# Autodesk Inventor assembly: Lick
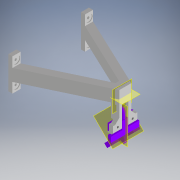
[picture p0: Inventor's stored thumbnail of the model, 180x180]
Saved by Autodesk Inventor 2020 (Build 240168000, 168)
## iProperties
Created: 2020-01-13
Part Number: Lick
Document SubType Name: Assembly
Designer: Knowblesse
Author: Knowblesse
## Documents named in this file (3)
- C:\VCF\Lobster\Apparatus\Lick\Lick.iam
- C:\VCF\Lobster\Apparatus\Lick\LickSensorMount_H.ipt
- C:\VCF\Lobster\Apparatus\Lick\LickModuleMount.ipt
## Components (2 placed, 2 different names)
1. LickSensorMount_H:1 — 강체:1
2. LickModuleMount:1 — 강체:1
## Relationships (1: WeldJoint 1)
- 강체:1 [WeldJoint]: LickSensorMount_H:1 ↔ LickModuleMount:1
